# Autodesk Inventor assembly: cameramount3.0
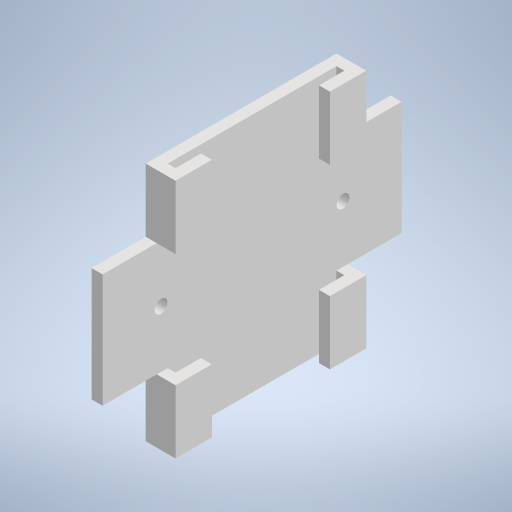
[picture p0: Inventor's stored thumbnail of the model, 512x512]
Saved by Autodesk Inventor 2024.3 (Build 283343000, 343)
## iProperties
Created: 2025-01-16
Part Number: cameramount3.0
Document SubType Name: Assembly
Designer: User
Author: User
## Documents named in this file (2)
- C:\Users\User\Desktop\BoardAndTiles\camera_mount\cameramount3.0.iam
- C:\Users\User\Desktop\BoardAndTiles\camera_mount\cam_holder3.ipt
## Components (2 placed, 1 different names)
1. cam_holder3:1 — Mate:1, Mate:2
2. cam_holder3:2 — Mate:1, Mate:2
## Relationships (2: Mate 2)
- Mate:1: cam_holder3:1 ↔ cam_holder3:2
- Mate:2: cam_holder3:1 ↔ cam_holder3:2
